# Autodesk Inventor assembly: TL20240701-10200AT-000
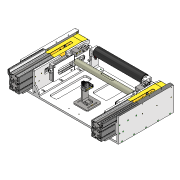
[picture p0: Inventor's stored thumbnail of the model, 180x180]
Saved by Autodesk Inventor 2022.5 (Build 265521000, 521)
## iProperties
Category: CONVEYOR ASSY
Company: 현대트랜시스(대유)
RuleStatus: InUse
Created: 2024-07-26
Part Number: TL20240701-10200AT-000
Project: SW-PJT
Checked By: 김형민
Engr Approved By: 김시현
User Status: 1 x13
Material: SS400
Description: 5
Document SubType Name: Assembly
Mfg Approved By: 호상태
Designer: USER106
Stock Number: 000
Mass: 3528.01 g
Surface Area: 796.864 cm^2
Volume: 469.444 cm^3
Density: 7.5153 g/cm^3
Deteil Description: Detail Description
Detail Description: Assembly products
Title: ANTI BACK ASSY
Subject: SW차종 시트조립라인
Author: USER106
Revision Number: A
## Documents named in this file (12)
- D:\V\Designs\프로젝트 자산\자동화 & 스마트팩토리\현대트랜시스(구 다이모스, 파워텍)\현대트랜시스(대유화성공장)_SW 시트조립라인\2.제작도면\1. 1ST LINE\ANTI BACK\TL20240701-10200AT\TL20240701-10200AT-000.iam
- D:\V\Designs\프로젝트 자산\자동화 & 스마트팩토리\현대트랜시스(구 다이모스, 파워텍)\현대트랜시스(대유화성공장)_SW 시트조립라인\2.제작도면\1. 1ST LINE\ANTI BACK\TL20240701-10200AT\TL20240701-10200AT-004.ipt
- D:\V\Designs\프로젝트 자산\자동화 & 스마트팩토리\현대트랜시스(구 다이모스, 파워텍)\현대트랜시스(대유화성공장)_SW 시트조립라인\2.제작도면\1. 1ST LINE\ANTI BACK\TL20240701-10200AT\TL20240701-10200AT-001.ipt
- D:\V\Designs\프로젝트 자산\자동화 & 스마트팩토리\현대트랜시스(구 다이모스, 파워텍)\현대트랜시스(대유화성공장)_SW 시트조립라인\2.제작도면\1. 1ST LINE\ANTI BACK\TL20240701-10200AT\TL20240701-10200AT-002.ipt
- D:\V\Designs\프로젝트 자산\자동화 & 스마트팩토리\현대트랜시스(구 다이모스, 파워텍)\현대트랜시스(대유화성공장)_SW 시트조립라인\2.제작도면\1. 1ST LINE\ANTI BACK\TL20240701-10200AT\TL20240701-10200AT-003.ipt
- D:\V\Designs\프로젝트 자산\자동화 & 스마트팩토리\현대트랜시스(구 다이모스, 파워텍)\현대트랜시스(대유화성공장)_SW 시트조립라인\2.제작도면\기타(도면용 구성품)\PROFILE_Simplify-B.ipt
- D:\V\Designs\구매품(업체별)\LUBO\DU BUSH_MB0808-15FDU_LUBO.ipt
- D:\V\Content Center Files\en-US\KS B 1320  A\KS B 1320 - A 3 x  16.ipt
- D:\V\Content Center Files\en-US\KS B 1012  C\KS B 1012 - C M8C.ipt
- D:\V\Designs\프로젝트 자산\자동화 & 스마트팩토리\현대트랜시스(구 다이모스, 파워텍)\현대트랜시스(대유화성공장)_SW 시트조립라인\2.제작도면\기타(도면용 구성품)\1열\TL20240701-10120CV-000_Simplify.ipt
- D:\V\Designs\프로젝트 자산\자동화 & 스마트팩토리\현대트랜시스(구 다이모스, 파워텍)\현대트랜시스(대유화성공장)_SW 시트조립라인\2.제작도면\1. 1ST LINE\ANTI BACK\TL20240701-10200AT\TL20240701-10200AT-005.ipt
- D:\V\Content Center Files\en-US\KS B 1003\KS B 1003 - M 8 x 35.ipt
## Components (12 placed, 11 different names)
1. DU BUSH_MB0808-15FDU_LUBO.ipt:1
2. DU BUSH_MB0808-15FDU_LUBO.ipt:2
3. KS B 1003 - M 8 x 35.ipt:1
4. KS B 1012 - C M8C.ipt:1
5. KS B 1320 - A 3 x  16.ipt:1
6. PROFILE_Simplify-B.ipt:1 — Mate:39, Flush:8, Mate:49, Mate:50, Mate:51, Mate:66
7. TL20240701-10120CV-000_Simplify.ipt:1 — Mate:49, Mate:50, Mate:51, Mate:52, Mate:67, Flush:13
8. TL20240701-10200AT-001.ipt:1 — Mate:66, Mate:68, Mate:70, Flush:15
9. TL20240701-10200AT-002.ipt:1
10. TL20240701-10200AT-003.ipt:1
11. TL20240701-10200AT-004.ipt:1 — Mate:30, Mate:39, Flush:8, Mate:67, Mate:68, Mate:69, Mate:73, Flush:14
12. TL20240701-10200AT-005.ipt:1 — Mate:69, Mate:70, Mate:73, Flush:14, Flush:15
## Relationships (33: Mate 25, Flush 7, Angle 1)
- Mate:30: TL20240701-10200AT-004.ipt:1
- Mate:39 (242 mm): PROFILE_Simplify-B.ipt:1 ↔ TL20240701-10200AT-004.ipt:1
- Flush:8 (49 mm): PROFILE_Simplify-B.ipt:1 ↔ TL20240701-10200AT-004.ipt:1
- Mate:49: PROFILE_Simplify-B.ipt:1 ↔ TL20240701-10120CV-000_Simplify.ipt:1
- Mate:50: PROFILE_Simplify-B.ipt:1 ↔ TL20240701-10120CV-000_Simplify.ipt:1
- Mate:51: PROFILE_Simplify-B.ipt:1 ↔ TL20240701-10120CV-000_Simplify.ipt:1
- Mate:52: TL20240701-10120CV-000_Simplify.ipt:1
- [Mate]: TL20240701-10200AT-001.ipt:1 ↔ TL20240701-10200AT-002.ipt:1
- [Flush]: TL20240701-10200AT-001.ipt:1 ↔ TL20240701-10200AT-002.ipt:1
- [Mate]: TL20240701-10200AT-002.ipt:1 ↔ TL20240701-10200AT-003.ipt:1
- [Mate] (1 mm): TL20240701-10200AT-001.ipt:1 ↔ TL20240701-10200AT-003.ipt:1
- [Angle] (0 deg): TL20240701-10200AT-001.ipt:1 ↔ TL20240701-10200AT-003.ipt:1
- [Mate]: TL20240701-10200AT-001.ipt:1 ↔ TL20240701-10200AT-003.ipt:1
- [Mate]: KS B 1003 - M 8 x 35.ipt:1 ↔ TL20240701-10200AT-003.ipt:1
- [Flush]: KS B 1003 - M 8 x 35.ipt:1 ↔ TL20240701-10200AT-003.ipt:1
- [Mate]: KS B 1003 - M 8 x 35.ipt:1 ↔ KS B 1012 - C M8C.ipt:1
- [Mate]: KS B 1012 - C M8C.ipt:1 ↔ TL20240701-10200AT-003.ipt:1
- [Mate]: DU BUSH_MB0808-15FDU_LUBO.ipt:1 ↔ TL20240701-10200AT-002.ipt:1
- [Mate]: DU BUSH_MB0808-15FDU_LUBO.ipt:1 ↔ TL20240701-10200AT-001.ipt:1
- [Mate]: DU BUSH_MB0808-15FDU_LUBO.ipt:2 ↔ TL20240701-10200AT-002.ipt:1
- [Mate]: DU BUSH_MB0808-15FDU_LUBO.ipt:2 ↔ TL20240701-10200AT-001.ipt:1
- [Mate]: KS B 1320 - A 3 x  16.ipt:1 ↔ TL20240701-10200AT-001.ipt:1
- [Flush]: KS B 1320 - A 3 x  16.ipt:1 ↔ TL20240701-10200AT-001.ipt:1
- [Mate]: TL20240701-10200AT-001.ipt:1 ↔ TL20240701-10200AT-003.ipt:1
- Mate:66: PROFILE_Simplify-B.ipt:1 ↔ TL20240701-10200AT-001.ipt:1
- Mate:67: TL20240701-10120CV-000_Simplify.ipt:1 ↔ TL20240701-10200AT-004.ipt:1
- Flush:13: TL20240701-10120CV-000_Simplify.ipt:1
- Mate:68 (-17 mm): TL20240701-10200AT-001.ipt:1 ↔ TL20240701-10200AT-004.ipt:1
- Mate:69: TL20240701-10200AT-004.ipt:1 ↔ TL20240701-10200AT-005.ipt:1
- Mate:70: TL20240701-10200AT-001.ipt:1 ↔ TL20240701-10200AT-005.ipt:1
- Mate:73 (3.3 mm): TL20240701-10200AT-004.ipt:1 ↔ TL20240701-10200AT-005.ipt:1
- Flush:14 (35 mm): TL20240701-10200AT-004.ipt:1 ↔ TL20240701-10200AT-005.ipt:1
- Flush:15 (7.5 mm): TL20240701-10200AT-001.ipt:1 ↔ TL20240701-10200AT-005.ipt:1
